# Autodesk Inventor assembly: body_base
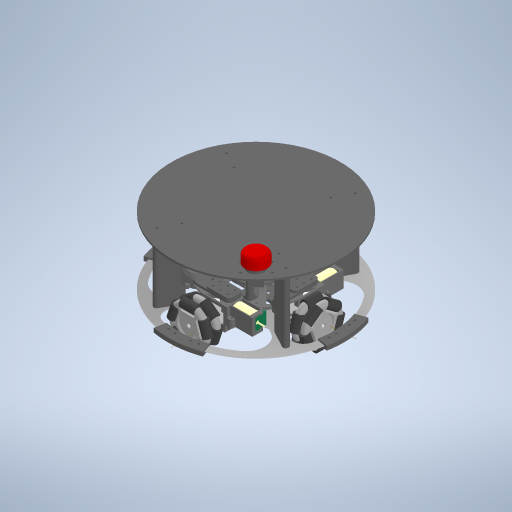
[picture p0: Inventor's stored thumbnail of the model, 512x512]
Saved by Autodesk Inventor 2024.1 (Build 281209000, 209)
## iProperties
Created: 2024-08-02
Part Number: body_base
Document SubType Name: Assembly
Designer: hibik
Author: hibik
## Documents named in this file (9)
- C:\Users\hibik\Desktop\ロボメカ\Rescue\2年\子機_本選\body_base.iam
- C:\Users\hibik\Desktop\ロボメカ\Rescue\2年\子機_本選\board_base_connect.ipt
- C:\Users\hibik\Desktop\ロボメカ\Rescue\2年\子機_本選\body_locom.iam
- C:\Users\hibik\Desktop\ロボメカ\Rescue\2年\子機_本選\plate_cover.ipt
- C:\Users\hibik\Desktop\ロボメカ\Rescue\2年\子機_本選\battery_cover.ipt
- C:\Users\hibik\Desktop\ロボメカ\Rescue\2年\子機_本選\upper_plate.ipt
- C:\Users\hibik\Desktop\ロボメカ\Rescue\2年\子機_本選\pole.ipt
- C:\Users\hibik\Desktop\ロボメカ\Rescue\2年\子機_本選\emergency_button.ipt
- C:\Users\hibik\Desktop\ロボメカ\Rescue\2年\子機_本選\board_set.iam
## Components (14 placed, 8 different names)
1. board_base_connect:1 — 挿入:5, 挿入:6, 挿入:29, 挿入:30
2. body_locom:1 [sub-assembly] — 挿入:5, 挿入:6, 挿入:7, 挿入:9, 挿入:10, 挿入:11, 挿入:12, 挿入:13, 挿入:14, 挿入:15, 挿入:16, 挿入:17, 挿入:18, 挿入:19, 挿入:23, 挿入:24, 挿入:25, 挿入:26, 挿入:27, 挿入:28
3. plate_cover:1 — 挿入:7, 挿入:13
4. plate_cover:3 — 挿入:9, 挿入:12
5. plate_cover:4 — 挿入:10, 挿入:11
6. plate_cover:5 — 挿入:14, 挿入:15
7. battery_cover:1 — 挿入:16, 挿入:17
8. pole:1 — 挿入:18, 挿入:19, 挿入:20, 挿入:21
9. upper_plate:2 — 挿入:20, 挿入:21, 挿入:22
10. emergency_button:1 — 挿入:22
11. pole:2 — 挿入:23, 挿入:27
12. pole:3 — 挿入:24, 挿入:28
13. pole:4 — 挿入:25, 挿入:26
14. board_set:1 [sub-assembly] — 挿入:29, 挿入:30
## Relationships (25: Insert 25)
- 挿入:5 [Insert]: board_base_connect:1 ↔ body_locom:1
- 挿入:6 [Insert]: board_base_connect:1 ↔ body_locom:1
- 挿入:7 [Insert]: body_locom:1 ↔ plate_cover:1
- 挿入:9 [Insert]: body_locom:1 ↔ plate_cover:3
- 挿入:10 [Insert]: body_locom:1 ↔ plate_cover:4
- 挿入:11 [Insert]: body_locom:1 ↔ plate_cover:4
- 挿入:12 [Insert]: body_locom:1 ↔ plate_cover:3
- 挿入:13 [Insert]: body_locom:1 ↔ plate_cover:1
- 挿入:14 [Insert]: body_locom:1 ↔ plate_cover:5
- 挿入:15 [Insert]: body_locom:1 ↔ plate_cover:5
- 挿入:16 [Insert]: body_locom:1 ↔ battery_cover:1
- 挿入:17 [Insert]: body_locom:1 ↔ battery_cover:1
- 挿入:18 [Insert]: body_locom:1 ↔ pole:1
- 挿入:19 [Insert]: body_locom:1 ↔ pole:1
- 挿入:20 [Insert]: pole:1 ↔ upper_plate:2
- 挿入:21 [Insert]: pole:1 ↔ upper_plate:2
- 挿入:22 [Insert]: upper_plate:2 ↔ emergency_button:1
- 挿入:23 [Insert]: body_locom:1 ↔ pole:2
- 挿入:24 [Insert]: body_locom:1 ↔ pole:3
- 挿入:25 [Insert]: body_locom:1 ↔ pole:4
- 挿入:26 [Insert]: body_locom:1 ↔ pole:4
- 挿入:27 [Insert]: body_locom:1 ↔ pole:2
- 挿入:28 [Insert]: body_locom:1 ↔ pole:3
- 挿入:29 [Insert]: board_base_connect:1 ↔ board_set:1
- 挿入:30 [Insert]: board_base_connect:1 ↔ board_set:1
